# Autodesk Inventor assembly: Head
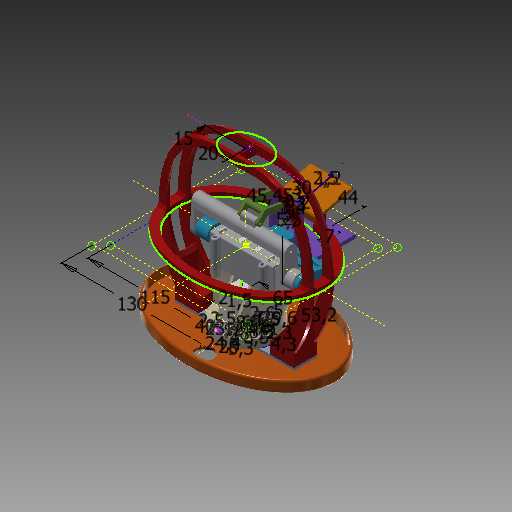
[picture p0: Inventor's stored thumbnail of the model, 512x512]
Saved by Autodesk Inventor 2018.3 (Build 223284000, 284)
## iProperties
Created: 2018-05-16
Part Number: Head
Material: Generisch
Document SubType Name: Assembly
Designer: JochenAlt
Author: JochenAlt
## Documents named in this file (14)
- D:\Projects\Donna\CAD\Head.iam
- D:\Projects\Donna\CAD\Stewart-Head.ipt
- D:\Projects\Donna\CAD\Mouth-Base.ipt
- D:\Projects\Donna\CAD\Servo-KST-DS215MG.ipt
- D:\Projects\Donna\CAD\Rillenkugellager 61707-2RS1.iam
- D:\Projects\Donna\CAD\Mouth-Height-Lever-front.ipt
- D:\Projects\Donna\CAD\Ball-Joint-male.ipt
- D:\Projects\Donna\CAD\Servo-Arm-Lip.ipt
- D:\Projects\Donna\CAD\Servo-Arm-Mouth.ipt
- C:\Users\JochenAlt\Documents\Inventor\Content Center Files\R2018\de-DE\BS 290 SKF(30)\BS 290 SKF - SKF 623.ipt
- D:\Projects\Donna\CAD\Mouth-Turn-Disk.ipt
- D:\Projects\Donna\CAD\Mouth-Height-Lever.ipt
- D:\Projects\Donna\CAD\Mouth-Upper-Holder.ipt
- D:\Projects\Donna\CAD\Bottom-Lip.ipt
## Components (21 placed, 10 different names)
1. Stewart-Plate-Head:1 — Passend:3, Passend:6, Passend:7, Passend:18, Passend:19, Passend:20, Passend:21, Passend:22, Passend:23, Passend:24, Passend:25, Passend:26, Passend:27, Passend:28, Passend:29, Passend:88, Passend:89, Passend:90, Passend:95
2. Mouth-Base:1 — Passend:60, Passend:61, Passend:72, Passend:73, Passend:96, Passend:102, Passend:103, Passend:104, Passend:105
3. Servo-KST-DS215MG:1 — Passend:3, Passend:105
4. Rillenkugellager 61707-2RS1:1 [sub-assembly] — Passend:6, Passend:7, Passend:96, Passend:103
5. Mouth-Height-Lever:2 — Passend:69, Passend:70, Passend:80, Passend:81, Passend:86
6. ball joint:1 — Passend:18, Passend:29
7. ball joint:2 — Passend:19, Passend:28
8. ball joint:3 — Passend:23, Passend:25
9. ball joint:4 — Passend:22, Passend:24
10. ball joint:5 — Passend:21, Passend:27
11. ball joint:6 — Passend:20, Passend:26
12. Servo-KST-DS215MG:2 — Passend:38, Passend:39, Passend:61, Passend:73, Passend:104
13. Servo-KST-DS215MG:3 — Passend:37, Passend:60, Passend:68, Passend:72, Passend:102
14. ServoArm:1 — Passend:37, Passend:40, Passend:41, Passend:68, Passend:80
15. ServoArm:2 — Passend:38, Passend:39, Passend:44, Passend:45, Passend:71, Passend:85
16. BS 290 SKF 623:1 — Passend:40, Passend:41
17. BS 290 SKF 623:2 — Passend:44, Passend:45
18. Mouth-Turn-Disk:1 — Passend:95
19. Mouth-Height-Lever:3 — Passend:69, Passend:70, Passend:71, Passend:81, Passend:85, Passend:86
20. Mouth-Height-Lever:4 — Passend:88, Passend:89, Passend:90, Passend:100, Passend:101
21. Bottom-Lip:1 — Passend:100, Passend:101
## Relationships (45: Mate 45)
- Passend:3 [Mate]: Stewart-Plate-Head:1 ↔ Servo-KST-DS215MG:1
- Passend:6 [Mate]: Stewart-Plate-Head:1 ↔ Rillenkugellager 61707-2RS1:1
- Passend:7 [Mate]: Stewart-Plate-Head:1 ↔ Rillenkugellager 61707-2RS1:1
- Passend:18 [Mate]: Stewart-Plate-Head:1 ↔ ball joint:1
- Passend:19 [Mate]: Stewart-Plate-Head:1 ↔ ball joint:2
- Passend:20 [Mate]: Stewart-Plate-Head:1 ↔ ball joint:6
- Passend:21 [Mate]: Stewart-Plate-Head:1 ↔ ball joint:5
- Passend:22 [Mate]: Stewart-Plate-Head:1 ↔ ball joint:4
- Passend:23 [Mate]: Stewart-Plate-Head:1 ↔ ball joint:3
- Passend:24 [Mate]: Stewart-Plate-Head:1 ↔ ball joint:4
- Passend:25 [Mate]: Stewart-Plate-Head:1 ↔ ball joint:3
- Passend:26 [Mate]: Stewart-Plate-Head:1 ↔ ball joint:6
- Passend:27 [Mate]: Stewart-Plate-Head:1 ↔ ball joint:5
- Passend:28 [Mate]: Stewart-Plate-Head:1 ↔ ball joint:2
- Passend:29 [Mate]: Stewart-Plate-Head:1 ↔ ball joint:1
- Passend:37 [Mate] (3.1 mm): Servo-KST-DS215MG:3 ↔ ServoArm:1
- Passend:38 [Mate]: Servo-KST-DS215MG:2 ↔ ServoArm:2
- Passend:39 [Mate] (3.1 mm): Servo-KST-DS215MG:2 ↔ ServoArm:2
- Passend:40 [Mate]: ServoArm:1 ↔ BS 290 SKF 623:1
- Passend:41 [Mate]: ServoArm:1 ↔ BS 290 SKF 623:1
- Passend:44 [Mate]: ServoArm:2 ↔ BS 290 SKF 623:2
- Passend:45 [Mate]: ServoArm:2 ↔ BS 290 SKF 623:2
- Passend:60 [Mate]: Mouth-Base:1 ↔ Servo-KST-DS215MG:3
- Passend:61 [Mate]: Mouth-Base:1 ↔ Servo-KST-DS215MG:2
- Passend:68 [Mate]: Servo-KST-DS215MG:3 ↔ ServoArm:1
- Passend:69 [Mate]: Mouth-Height-Lever:2 ↔ Mouth-Height-Lever:3
- Passend:70 [Mate] (0.5 mm): Mouth-Height-Lever:2 ↔ Mouth-Height-Lever:3
- Passend:71 [Mate]: ServoArm:2 ↔ Mouth-Height-Lever:3
- Passend:72 [Mate]: Mouth-Base:1 ↔ Servo-KST-DS215MG:3
- Passend:73 [Mate]: Mouth-Base:1 ↔ Servo-KST-DS215MG:2
- Passend:80 [Mate]: Mouth-Height-Lever:2 ↔ ServoArm:1
- Passend:81 [Mate]: Mouth-Height-Lever:2 ↔ Mouth-Height-Lever:3
- Passend:85 [Mate] (0.5 mm): ServoArm:2 ↔ Mouth-Height-Lever:3
- Passend:86 [Mate] (0.5 mm): Mouth-Height-Lever:2 ↔ Mouth-Height-Lever:3
- Passend:88 [Mate]: Stewart-Plate-Head:1 ↔ Mouth-Height-Lever:4
- Passend:89 [Mate]: Stewart-Plate-Head:1 ↔ Mouth-Height-Lever:4
- Passend:90 [Mate]: Stewart-Plate-Head:1 ↔ Mouth-Height-Lever:4
- Passend:95 [Mate]: Stewart-Plate-Head:1 ↔ Mouth-Turn-Disk:1
- Passend:96 [Mate]: Mouth-Base:1 ↔ Rillenkugellager 61707-2RS1:1
- Passend:100 [Mate]: Mouth-Height-Lever:4 ↔ Bottom-Lip:1
- Passend:101 [Mate] (0.5 mm): Mouth-Height-Lever:4 ↔ Bottom-Lip:1
- Passend:102 [Mate]: Mouth-Base:1 ↔ Servo-KST-DS215MG:3
- Passend:103 [Mate]: Mouth-Base:1 ↔ Rillenkugellager 61707-2RS1:1
- Passend:104 [Mate]: Mouth-Base:1 ↔ Servo-KST-DS215MG:2
- Passend:105 [Mate]: Mouth-Base:1 ↔ Servo-KST-DS215MG:1
